# Autodesk Inventor assembly: Assembly1
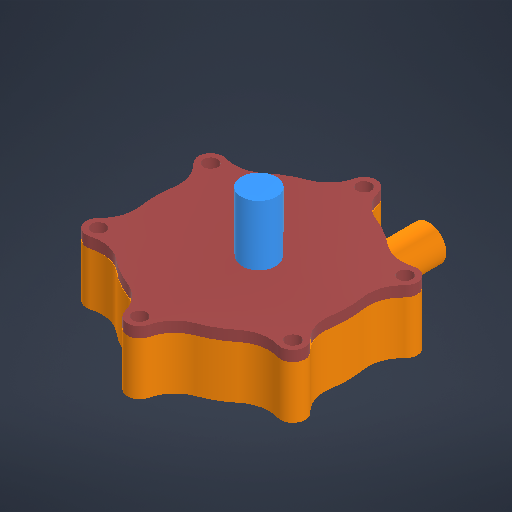
[picture p0: Inventor's stored thumbnail of the model, 512x512]
Saved by Autodesk Inventor 2025.3 (Build 293356000, 356)
## iProperties
Created: 2025-10-02
Part Number: Assembly1
Document SubType Name: Assembly
Designer: sophi
Author: sophi
## Documents named in this file (6)
- C:\Users\sophi\OneDrive - Universidad de los andes\Documentos\1 Universidad\5 Semestre\Proyecto\Vane\Assembly1.iam
- C:\Users\sophi\OneDrive - Universidad de los andes\Documentos\1 Universidad\5 Semestre\Proyecto\Vane\carcaza motor.ipt
- C:\Users\sophi\OneDrive - Universidad de los andes\Documentos\1 Universidad\5 Semestre\Proyecto\Vane\intermo.ipt
- C:\Users\sophi\OneDrive - Universidad de los andes\Documentos\1 Universidad\5 Semestre\Proyecto\Vane\paletas.ipt
- C:\Users\sophi\OneDrive - Universidad de los andes\Documentos\1 Universidad\5 Semestre\Proyecto\Vane\rodamiento.ipt
- C:\Users\sophi\OneDrive - Universidad de los andes\Documentos\1 Universidad\5 Semestre\Proyecto\Vane\tapa.ipt
## Components (6 placed, 5 different names)
1. carcaza motor:1 — Flush:1, Flush:2, Flush:3, Insert:1, Tangent:1, Flush:4, Mate:8
2. intermo:1 — Mate:2, Mate:3, Mate:5, Mate:7
3. paletas:1 — Mate:1, Mate:2, Tangent:1, Mate:6
4. rodamiento:1 — Mate:1, Insert:1, Mate:3
5. rodamiento:2 — Mate:5, Mate:6
6. tapa:1 — Flush:4, Mate:7, Mate:8
## Relationships (13: Mate 7, Flush 4, Insert 1, Tangent 1)
- Flush:1: carcaza motor:1
- Flush:2: carcaza motor:1
- Flush:3: carcaza motor:1
- Mate:1: paletas:1 ↔ rodamiento:1
- Insert:1: carcaza motor:1 ↔ rodamiento:1
- Mate:2: intermo:1 ↔ paletas:1
- Mate:3: intermo:1 ↔ rodamiento:1
- Tangent:1: carcaza motor:1 ↔ paletas:1
- Mate:5: intermo:1 ↔ rodamiento:2
- Mate:6: paletas:1 ↔ rodamiento:2
- Flush:4: carcaza motor:1 ↔ tapa:1
- Mate:7: intermo:1 ↔ tapa:1
- Mate:8: carcaza motor:1 ↔ tapa:1
